# Autodesk Inventor assembly: SM_YA01
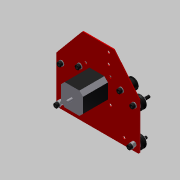
[picture p0: Inventor's stored thumbnail of the model, 180x180]
Saved by Autodesk Inventor 2013 (Build 170138000, 138)
## iProperties
Created: 2012-05-01
Part Number: SM_YA01
Document SubType Name: Assembly
Designer: ERF
Stock Number: SM_YA01
Author: ERF
Title: Y Axis Motor Mount Assembly
## Documents named in this file (13)
- C:\Users\Brett\Documents\Autodesk\Projects\Shapeoko_v1i\Assemblies\SM-YA01.iam
- C:\Users\Brett\Documents\Autodesk\Projects\Shapeoko_v1i\Parts\MSK01-09.ipt
- C:\Users\Brett\Documents\Autodesk\Projects\Shapeoko_v1i\Parts\SM-E01.ipt
- C:\Users\Brett\Documents\Autodesk\Projects\Shapeoko_v1i\Parts\SM-S01.ipt
- C:\Users\Brett\Documents\Autodesk\Projects\Shapeoko_v1i\Parts\SM-H04.ipt
- C:\Users\Brett\Documents\Autodesk\Projects\Shapeoko_v1i\Parts\SM-H01.ipt
- C:\Users\Brett\Documents\Autodesk\Projects\Shapeoko_v1i\Parts\SM-H08.ipt
- C:\Users\Brett\Documents\Autodesk\Projects\Shapeoko_v1i\Parts\MSK01-04.ipt
- C:\Users\Brett\Documents\Autodesk\Projects\Shapeoko_v1i\Parts\SM-H03.ipt
- C:\Users\Brett\Documents\Autodesk\Projects\Shapeoko_v1i\Parts\SM-H14.ipt
- C:\Users\Brett\Documents\Autodesk\Projects\Shapeoko_v1i\Parts\SM-H15.ipt
- C:\Users\Brett\Documents\Autodesk\Projects\Shapeoko_v1i\Assemblies\MSK01-05A.iam
- C:\Users\Brett\Documents\Autodesk\Projects\Shapeoko_v1i\Assemblies\MSK01-06A.iam
## Components (53 placed, 12 different names)
1. MSK01-09:1 — Insert:43
2. SM-E01:1 — Insert:42, Angle:1, Insert:43
3. SM-S01:1 — Insert:9, Insert:10, Insert:11, Insert:12, Insert:13, Insert:14, Mate:2, Mate:4, Insert:27, Insert:28, Insert:29, Insert:30, Insert:42, Angle:1, Insert:48, Insert:49, Insert:50, Insert:51
4. SM-H01:1 — Insert:31, Insert:35
5. MSK01-05A:5 [sub-assembly] — Insert:54, Insert:55
6. SM-H08:1 — Insert:1
7. SM-H04:2 — Insert:23
8. SM-H08:2 — Insert:2
9. MSK01-05A:6 [sub-assembly] — Insert:57, Insert:60
10. SM-H04:3 — Insert:24
11. SM-H08:3 — Insert:3, Insert:7, Mate:1
12. MSK01-04:1 — Insert:7, Insert:11
13. SM-H08:4 — Insert:4
14. SM-H04:4 — Insert:25
15. MSK01-05A:7 [sub-assembly] — Insert:56, Insert:61
16. SM-H08:5 — Insert:5
17. SM-H01:2 — Insert:33, Insert:34
18. SM-H04:5 — Insert:26
19. MSK01-04:2 — Insert:8, Insert:12
20. SM-H08:6 — Insert:6, Mate:3
21. MSK01-05A:8 [sub-assembly] — Insert:58, Insert:59
22. SM-H03:2 — Insert:6, Insert:8
23. SM-H03:3 — Insert:5, Insert:28
24. SM-H03:4 — Insert:4, Insert:27
25. SM-H03:5 — Insert:3
26. SM-H03:6 — Insert:2, Insert:10
27. SM-H03:7 — Insert:1, Insert:9
28. SM-H03:8 — Insert:13, Insert:59
29. SM-H03:9 — Mate:3, Mate:4, Insert:55
30. SM-H03:10 — Insert:24, Insert:56
31. SM-H03:11 — Insert:14, Insert:61
32. SM-H03:12 — Insert:30, Insert:31
33. SM-H03:14 — Insert:34, Insert:62
34. SM-H03:15 — Insert:25, Insert:57
35. SM-H03:16 — Insert:26, Insert:54
36. SM-H03:17 — Insert:23, Insert:58
37. SM-H03:18 — Insert:29, Insert:33
38. SM-H03:19 — Mate:1, Mate:2, Insert:60
39. SM-H03:20 — Insert:40, Insert:64
40. SM-H04:6 — Insert:41
41. SM-H03:21 — Insert:41, Insert:65
42. SM-H04:7 — Insert:40
43. SM-H03:22 — Insert:35, Insert:63
44. SM-H14:1 — Insert:44
45. SM-H15:1 — Insert:44, Insert:51
46. SM-H14:2 — Insert:45
47. SM-H15:2 — Insert:45, Insert:50
48. SM-H14:3 — Insert:46
49. SM-H15:3 — Insert:46, Insert:49
50. SM-H14:4 — Insert:47
51. SM-H15:4 — Insert:47, Insert:48
52. MSK01-06A:6 [sub-assembly] — Insert:62, Insert:65
53. MSK01-06A:7 [sub-assembly] — Insert:63, Insert:64
## Relationships (55: Insert 50, Mate 4, Angle 1)
- Insert:1: SM-H08:1 ↔ SM-H03:7
- Insert:2: SM-H08:2 ↔ SM-H03:6
- Insert:3: SM-H08:3 ↔ SM-H03:5
- Insert:4: SM-H08:4 ↔ SM-H03:4
- Insert:5: SM-H08:5 ↔ SM-H03:3
- Insert:6: SM-H08:6 ↔ SM-H03:2
- Insert:7: SM-H08:3 ↔ MSK01-04:1
- Insert:8: MSK01-04:2 ↔ SM-H03:2
- Insert:9: SM-S01:1 ↔ SM-H03:7
- Insert:10: SM-S01:1 ↔ SM-H03:6
- Insert:11: SM-S01:1 ↔ MSK01-04:1
- Insert:12: SM-S01:1 ↔ MSK01-04:2
- Insert:13: SM-S01:1 ↔ SM-H03:8
- Insert:14: SM-S01:1 ↔ SM-H03:11
- Mate:1: SM-H08:3 ↔ SM-H03:19
- Mate:2: SM-S01:1 ↔ SM-H03:19
- Mate:3: SM-H08:6 ↔ SM-H03:9
- Mate:4: SM-S01:1 ↔ SM-H03:9
- Insert:23: SM-H04:2 ↔ SM-H03:17
- Insert:24: SM-H04:3 ↔ SM-H03:10
- Insert:25: SM-H04:4 ↔ SM-H03:15
- Insert:26: SM-H04:5 ↔ SM-H03:16
- Insert:27: SM-S01:1 ↔ SM-H03:4
- Insert:28: SM-S01:1 ↔ SM-H03:3
- Insert:29: SM-S01:1 ↔ SM-H03:18
- Insert:30: SM-S01:1 ↔ SM-H03:12
- Insert:31: SM-H01:1 ↔ SM-H03:12
- Insert:33: SM-H01:2 ↔ SM-H03:18
- Insert:34: SM-H01:2 ↔ SM-H03:14
- Insert:35: SM-H01:1 ↔ SM-H03:22
- Insert:40: SM-H03:20 ↔ SM-H04:7
- Insert:41: SM-H04:6 ↔ SM-H03:21
- Insert:42: SM-E01:1 ↔ SM-S01:1
- Angle:1 (0 deg): SM-E01:1 ↔ SM-S01:1
- Insert:43 (6.35 mm): MSK01-09:1 ↔ SM-E01:1
- Insert:44: SM-H14:1 ↔ SM-H15:1
- Insert:45: SM-H14:2 ↔ SM-H15:2
- Insert:46: SM-H14:3 ↔ SM-H15:3
- Insert:47: SM-H14:4 ↔ SM-H15:4
- Insert:48: SM-S01:1 ↔ SM-H15:4
- Insert:49: SM-S01:1 ↔ SM-H15:3
- Insert:50: SM-S01:1 ↔ SM-H15:2
- Insert:51: SM-S01:1 ↔ SM-H15:1
- Insert:54: MSK01-05A:5 ↔ SM-H03:16
- Insert:55: MSK01-05A:5 ↔ SM-H03:9
- Insert:56: MSK01-05A:7 ↔ SM-H03:10
- Insert:57: MSK01-05A:6 ↔ SM-H03:15
- Insert:58: MSK01-05A:8 ↔ SM-H03:17
- Insert:59: MSK01-05A:8 ↔ SM-H03:8
- Insert:60: MSK01-05A:6 ↔ SM-H03:19
- Insert:61: MSK01-05A:7 ↔ SM-H03:11
- Insert:62: SM-H03:14 ↔ MSK01-06A:6
- Insert:63: SM-H03:22 ↔ MSK01-06A:7
- Insert:64: SM-H03:20 ↔ MSK01-06A:7
- Insert:65: SM-H03:21 ↔ MSK01-06A:6
